# Autodesk Inventor assembly: v1.0
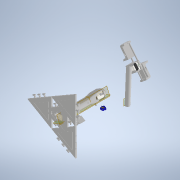
[picture p0: Inventor's stored thumbnail of the model, 180x180]
Saved by Autodesk Inventor 2022.3 (Build 263350000, 350)
## iProperties
Created: 2023-03-28
Part Number: v1.0
Document SubType Name: Assembly
Designer: Manuel Hueso Béjar
Author: Manuel Hueso Béjar
## Documents named in this file (18)
- C:\Users\Manuel Hueso Béjar\Desktop\3\2º Cuatrimestre\Robótica\2_Trabajo\CAD\v3.0\v2.0.iam
- C:\Users\Manuel Hueso Béjar\Desktop\3\2º Cuatrimestre\Robótica\2_Trabajo\CAD\v3.0\Base.ipt
- C:\Users\Manuel Hueso Béjar\Downloads\nema-17-motor-a-pasos-17hs4401-1-7amp-4kg-cm-1.snapshot.4\Nema 17 Motor a Pasos 17HS4401.iam
- C:\Users\Manuel Hueso Béjar\Desktop\3\2º Cuatrimestre\Robótica\2_Trabajo\CAD\v3.0\Base2.ipt
- C:\Users\Manuel Hueso Béjar\Desktop\3\2º Cuatrimestre\Robótica\2_Trabajo\CAD\v3.0\Tube_1_1.ipt
- C:\Users\Manuel Hueso Béjar\Desktop\3\2º Cuatrimestre\Robótica\2_Trabajo\CAD\v3.0\Tube_2.ipt
- C:\Users\Manuel Hueso Béjar\Desktop\3\2º Cuatrimestre\Robótica\2_Trabajo\CAD\v3.0\Joint_Tubes_1_2.ipt
- C:\Users\Manuel Hueso Béjar\Downloads\timing-pulley-gt2-16-teeth-5mm-bore-2.snapshot.7\GT2-16T\GT2_16T.ipt
- C:\Users\Manuel Hueso Béjar\Desktop\3\2º Cuatrimestre\Robótica\2_Trabajo\CAD\v3.0\Rod_1.ipt
- C:\Users\Manuel Hueso Béjar\Downloads\rolling-bearing-lmxxuu-1.snapshot.6\roulement lmxxuu (ap203).ipt
- C:\Users\Manuel Hueso Béjar\Desktop\3\2º Cuatrimestre\Robótica\2_Trabajo\CAD\v3.0\Joint_Bearings.ipt
- C:\Users\Manuel Hueso Béjar\Downloads\sg90-micro-servo-9g-tower-pro-1.snapshot.3\SG90 - Micro Servo 9g - Tower Pro.1.ipt
- C:\Users\Manuel Hueso Béjar\Desktop\3\2º Cuatrimestre\Robótica\2_Trabajo\CAD\v3.0\Tube_3.ipt
- C:\Users\Manuel Hueso Béjar\Desktop\3\2º Cuatrimestre\Robótica\2_Trabajo\CAD\v3.0\Potenciómetro_Roscado.ipt
- C:\Users\Manuel Hueso Béjar\Desktop\3\2º Cuatrimestre\Robótica\2_Trabajo\CAD\v3.0\Wire_Closing_1.ipt
- C:\Users\Manuel Hueso Béjar\Desktop\3\2º Cuatrimestre\Robótica\2_Trabajo\CAD\v3.0\Wire_Closing_2.ipt
- C:\Users\Manuel Hueso Béjar\Desktop\3\2º Cuatrimestre\Robótica\2_Trabajo\CAD\v3.0\Wire_Closing_3.ipt
- C:\Users\Manuel Hueso Béjar\Desktop\3\2º Cuatrimestre\Robótica\2_Trabajo\CAD\v3.0\Tube_1_2.ipt
## Components (24 placed, 17 different names)
1. Base:1 — Rotational:7, Rigid:27, Rigid:28, Rigid:29, Rotational:8, Rigid:31, Flush:1, Flush:2
2. Nema 17 Motor a Pasos 17HS4401:1 [sub-assembly] — Rotational:8
3. Tube_1_1:1 — Mate:3, Rigid:5, Mate:4, Mate:5, Mate:6, Mate:7, Rotational:7, Rigid:32
4. Tube_1_2:1 — Rigid:32
5. Nema 17 Motor a Pasos 17HS4401:2 [sub-assembly] — Mate:8, Mate:9, Mate:10, Rotational:6
6. Nema 17 Motor a Pasos 17HS4401:3 [sub-assembly] — Mate:3, Rigid:5, Rotational:2
7. Tube_2:1 — Rotational:6, Rigid:8
8. Joint_Tubes_1_2:1 — Mate:4, Rotational:3, Rotational:4
9. GT2_16T:1 — Rotational:2
10. Joint_Tubes_1_2:2 — Mate:5, Mate:6, Mate:7, Rotational:5
11. Rod_1:1 — Rotational:4, Cylindrical:2
12. Rod_1:2 — Rotational:3, Rotational:5, Cylindrical:1
13. roulement lmxxuu (ap203):1 — Cylindrical:1, Rigid:7
14. roulement lmxxuu (ap203):2 — Cylindrical:2, Rigid:6
15. Joint_Bearings:1 — Rigid:6, Rigid:7, Mate:8, Mate:9, Mate:10
16. SG90 - Micro Servo 9g - Tower Pro.1:1
17. Tube_3:1 — Rigid:8
18. Base2:1 — Rigid:27
19. Base2:2 — Rigid:29
20. Base2:3 — Rigid:28
21. Potenciómetro_Roscado:1
22. Wire_Closing_1:1 — Rigid:30, Rigid:31
23. Wire_Closing_2:1 — Rigid:30
24. Wire_Closing_3:1 — Flush:1, Flush:2
## Relationships (29: WeldJoint 10, Mate 8, RevoluteJoint 7, CylindricalJoint 2, Flush 2)
- Mate:3: Tube_1_1:1 ↔ Nema 17 Motor a Pasos 17HS4401:3
- Rigid:5 [WeldJoint]: Tube_1_1:1 ↔ Nema 17 Motor a Pasos 17HS4401:3
- Rotational:2 [RevoluteJoint] (2.65 mm): Nema 17 Motor a Pasos 17HS4401:3 ↔ GT2_16T:1
- Mate:4: Tube_1_1:1 ↔ Joint_Tubes_1_2:1
- Mate:5: Tube_1_1:1 ↔ Joint_Tubes_1_2:2
- Mate:6: Tube_1_1:1 ↔ Joint_Tubes_1_2:2
- Mate:7: Tube_1_1:1 ↔ Joint_Tubes_1_2:2
- Rotational:3 [RevoluteJoint]: Joint_Tubes_1_2:1 ↔ Rod_1:2
- Rotational:4 [RevoluteJoint]: Joint_Tubes_1_2:1 ↔ Rod_1:1
- Rotational:5 [RevoluteJoint]: Joint_Tubes_1_2:2 ↔ Rod_1:2
- Cylindrical:1: Rod_1:2 ↔ roulement lmxxuu (ap203):1
- Cylindrical:2: Rod_1:1 ↔ roulement lmxxuu (ap203):2
- Rigid:6 [WeldJoint]: roulement lmxxuu (ap203):2 ↔ Joint_Bearings:1
- Rigid:7 [WeldJoint]: roulement lmxxuu (ap203):1 ↔ Joint_Bearings:1
- Mate:8: Nema 17 Motor a Pasos 17HS4401:2 ↔ Joint_Bearings:1
- Mate:9: Nema 17 Motor a Pasos 17HS4401:2 ↔ Joint_Bearings:1
- Mate:10: Nema 17 Motor a Pasos 17HS4401:2 ↔ Joint_Bearings:1
- Rotational:6 [RevoluteJoint]: Nema 17 Motor a Pasos 17HS4401:2 ↔ Tube_2:1
- Rigid:8 [WeldJoint]: Tube_2:1 ↔ Tube_3:1
- Rotational:7 [RevoluteJoint]: Base:1 ↔ Tube_1_1:1
- Rigid:27 [WeldJoint]: Base:1 ↔ Base2:1
- Rigid:28 [WeldJoint]: Base:1 ↔ Base2:3
- Rigid:29 [WeldJoint]: Base:1 ↔ Base2:2
- Rotational:8 [RevoluteJoint]: Base:1 ↔ Nema 17 Motor a Pasos 17HS4401:1
- Rigid:30 [WeldJoint]: Wire_Closing_1:1 ↔ Wire_Closing_2:1
- Rigid:31 [WeldJoint]: Base:1 ↔ Wire_Closing_1:1
- Flush:1: Base:1 ↔ Wire_Closing_3:1
- Flush:2: Base:1 ↔ Wire_Closing_3:1
- Rigid:32 [WeldJoint]: Tube_1_1:1 ↔ Tube_1_2:1
